# Autodesk Inventor assembly: magnetometer_holder-asm
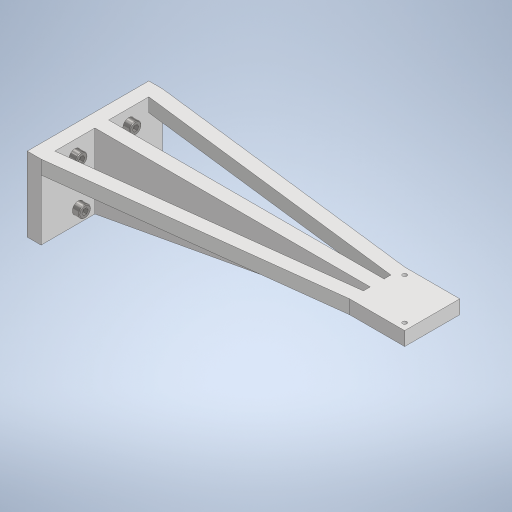
[picture p0: Inventor's stored thumbnail of the model, 512x512]
Saved by Autodesk Inventor 2024 (Build 280153000, 153)
## iProperties
Created: 2026-01-01
Part Number: magnetometer_holder-asm
Document SubType Name: Assembly
Designer: schar
Author: schar
## Documents named in this file (4)
- C:\Users\schar\Desktop\projectBlueprint\AMSTS\hardware\magnetometer_holder-asm.iam
- C:\Users\schar\Desktop\projectBlueprint\AMSTS\hardware\magnetometer_holder.ipt
- C:\Users\schar\Desktop\projectBlueprint\AMSTS\hardware\tnut_m5_2020.ipt
- C:\Users\schar\Documents\Inventor\Content Center Files\R2024\en-US\ISO 4762(1)\DIN EN ISO 4762 - M5 x 16.ipt
## Components (9 placed, 3 different names)
1. magnetometer_holder:1 — Rigid:1, Rigid:2, Rigid:3, Rigid:4, Mate:1, Mate:3, Mate:5, Mate:7
2. tnut_m5_2020:1 — Rigid:1, Mate:2
3. tnut_m5_2020:2 — Rigid:2, Mate:4
4. tnut_m5_2020:3 — Rigid:3, Mate:6
5. tnut_m5_2020:4 — Rigid:4, Mate:8
6. DIN EN ISO 4762 M5 x 16:1 — Mate:1, Mate:2
7. DIN EN ISO 4762 M5 x 16:2 — Mate:3, Mate:4
8. DIN EN ISO 4762 M5 x 16:3 — Mate:5, Mate:6
9. DIN EN ISO 4762 M5 x 16:4 — Mate:7, Mate:8
## Relationships (12: Mate 8, WeldJoint 4)
- Rigid:1 [WeldJoint] (0.159 mm): magnetometer_holder:1 ↔ tnut_m5_2020:1
- Rigid:2 [WeldJoint] (-0.159 mm): magnetometer_holder:1 ↔ tnut_m5_2020:2
- Rigid:3 [WeldJoint] (-0.159 mm): magnetometer_holder:1 ↔ tnut_m5_2020:3
- Rigid:4 [WeldJoint] (-0.159 mm): magnetometer_holder:1 ↔ tnut_m5_2020:4
- Mate:1: magnetometer_holder:1 ↔ DIN EN ISO 4762 M5 x 16:1
- Mate:2: tnut_m5_2020:1 ↔ DIN EN ISO 4762 M5 x 16:1
- Mate:3: magnetometer_holder:1 ↔ DIN EN ISO 4762 M5 x 16:2
- Mate:4: tnut_m5_2020:2 ↔ DIN EN ISO 4762 M5 x 16:2
- Mate:5: magnetometer_holder:1 ↔ DIN EN ISO 4762 M5 x 16:3
- Mate:6: tnut_m5_2020:3 ↔ DIN EN ISO 4762 M5 x 16:3
- Mate:7: magnetometer_holder:1 ↔ DIN EN ISO 4762 M5 x 16:4
- Mate:8: tnut_m5_2020:4 ↔ DIN EN ISO 4762 M5 x 16:4
